# Autodesk Inventor assembly: 276-2168
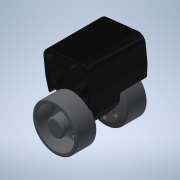
[picture p0: Inventor's stored thumbnail of the model, 180x180]
Saved by Autodesk Inventor 2020 (Build 240168000, 168)
## iProperties
Category: Motion
Company: Autodesk Inc.
Created: 2012-04-10
Part Number: 276-2168
Document SubType Name: Assembly
Designer: Autodesk Inc.
Catalog Web Link: http://www.vexrobotics.com/276-2168.html
Vendor: VEX
Author: Autodesk Inc.
## Documents named in this file (4)
- D:\Valut\ncrCadLib\链轮履带\Tank Drive Idler Single Wheel.iam
- D:\Valut\ncrCadLib\链轮履带\零件\IDLER-WHEEL-AXLE.ipt
- D:\Valut\ncrCadLib\链轮履带\零件\IDLER-WHEEL-ROLLER.ipt
- D:\Valut\ncrCadLib\链轮履带\零件\IDLER-WHEEL-SUPPORT.ipt
## Components (4 placed, 3 different names)
1. IDLER-WHEEL-AXLE — Mate:1, Mate:2, Mate:3, Mate:4, Mate:5, Mate:6
2. IDLER-WHEEL-ROLLER — Mate:1, Mate:2
3. IDLER-WHEEL-SUPPORT — Mate:5, Mate:6
4. IDLER-WHEEL-ROLLER — Mate:3, Mate:4
## Relationships (6: Mate 6)
- Mate:1: IDLER-WHEEL-AXLE ↔ IDLER-WHEEL-ROLLER
- Mate:2: IDLER-WHEEL-AXLE ↔ IDLER-WHEEL-ROLLER
- Mate:3: IDLER-WHEEL-AXLE ↔ IDLER-WHEEL-ROLLER
- Mate:4: IDLER-WHEEL-AXLE ↔ IDLER-WHEEL-ROLLER
- Mate:5: IDLER-WHEEL-AXLE ↔ IDLER-WHEEL-SUPPORT
- Mate:6: IDLER-WHEEL-AXLE ↔ IDLER-WHEEL-SUPPORT
